# Autodesk Inventor assembly: hubRingJig
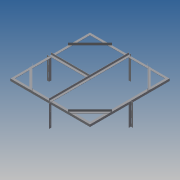
[picture p0: Inventor's stored thumbnail of the model, 180x180]
Saved by Autodesk Inventor 2014 SP1 (Build 180222100, 222)
## iProperties
Created: 2014-12-02
Part Number: hubRingJig
Document SubType Name: Assembly
Designer: Dave
Author: Dave
## Documents named in this file (6)
- C:\Users\Dave\Desktop\hera-cad\jigs\hubRingJig.iam
- C:\Users\Dave\Desktop\hera-cad\jigs\hubRingJigOuter.ipt
- C:\Users\Dave\Desktop\hera-cad\jigs\hubRingJigCross.ipt
- C:\Users\Dave\Desktop\hera-cad\jigs\hubRingJigEdgeVert.ipt
- C:\Users\Dave\Desktop\hera-cad\jigs\hubRingJigCrossShort.ipt
- C:\Users\Dave\Desktop\hera-cad\jigs\hubRingJig45.ipt
## Components (14 placed, 5 different names)
1. hubRingJigCross:1 — Mate:1, Flush:1, Flush:2, Flush:3, Mate:3, Flush:5, Flush:6
2. hubRingJigCrossShort:1 — Mate:3, Flush:5, Flush:6
3. hubRingJigOuter:1 — Mate:1, Flush:1, Flush:2, Mate:4, Flush:8
4. hubRingJigOuter:2 — Mate:2, Flush:4, Flush:7
5. hubRingJigOuter:3
6. hubRingJigOuter:4
7. hubRingJigEdgeVert:1 — Mate:2, Flush:3, Flush:4
8. hubRingJigEdgeVert:2
9. hubRingJigEdgeVert:3
10. hubRingJigEdgeVert:4
11. hubRingJig45:1 — Mate:4, Flush:7, Flush:8
12. hubRingJig45:2
13. hubRingJig45:3
14. hubRingJig45:4
## Component patterns: (4 elements, first: hubRingJigOuter:1), (4 elements, first: hubRingJigEdgeVert:1), (4 elements, first: hubRingJig45:1)
## Relationships (12: Flush 8, Mate 4)
- Mate:1: hubRingJigCross:1 ↔ hubRingJigOuter:1
- Flush:1 (-444.5 mm): hubRingJigCross:1 ↔ hubRingJigOuter:1
- Flush:2: hubRingJigCross:1 ↔ hubRingJigOuter:1
- Mate:2: hubRingJigOuter:2 ↔ hubRingJigEdgeVert:1
- Flush:3: hubRingJigCross:1 ↔ hubRingJigEdgeVert:1
- Flush:4: hubRingJigOuter:2 ↔ hubRingJigEdgeVert:1
- Mate:3: hubRingJigCross:1 ↔ hubRingJigCrossShort:1
- Flush:5: hubRingJigCross:1 ↔ hubRingJigCrossShort:1
- Flush:6 (-444.5 mm): hubRingJigCross:1 ↔ hubRingJigCrossShort:1
- Mate:4: hubRingJigOuter:1 ↔ hubRingJig45:1
- Flush:7: hubRingJigOuter:2 ↔ hubRingJig45:1
- Flush:8: hubRingJigOuter:1 ↔ hubRingJig45:1
